# Autodesk Inventor assembly: Ensamblaje completo
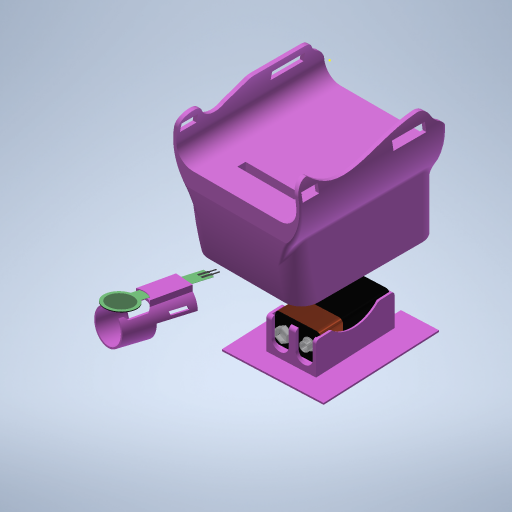
[picture p0: Inventor's stored thumbnail of the model, 512x512]
Saved by Autodesk Inventor 2024 (Build 280153000, 153)
## iProperties
Created: 2024-06-27
Part Number: Ensamblaje completo
Document SubType Name: Assembly
Designer: Valeria
Author: Valeria
## Documents named in this file (11)
- C:\Users\Valeria\Downloads\Ensamblaje completo.iam
- C:\Users\Valeria\Downloads\CASE batería.ipt
- C:\Users\Valeria\Downloads\9v-battery-11.snapshot.2\9v Duracell Battery Wyatt Sanders.ipt
- C:\Users\Valeria\Downloads\tapa ns (7).ipt
- C:\Users\Valeria\Downloads\coso tapa ns (3).ipt
- C:\Users\Valeria\Downloads\dedo ultimo xfa (1).ipt
- C:\Users\Valeria\Downloads\protoboard-400-pts-1.snapshot.5\proto_400\proto_400.ipt
- C:\Users\Valeria\Downloads\fsr402-1.snapshot.3\FSR 402\FSR 402.ipt
- C:\Users\Valeria\Downloads\arduino-nano-7.snapshot.2 (1)\arduino nano\arduino nano.ipt
- C:\Users\Valeria\Downloads\arduino-nano-7.snapshot.2 (1)\Green Detailed 5mm LED\Green Detailed 5mm LED.ipt
- C:\Users\Valeria\Downloads\arduino-nano-7.snapshot.2 (1)\Red Detailed 5mm LED\Red Detailed 5mm LED.ipt
## Components (10 placed, 10 different names)
1. CASE batería:1 — Coincidencia:1, Coincidencia:2, Coincidencia:3, Rígido:1
2. 9v Duracell Battery Wyatt Sanders:1 — Coincidencia:1, Coincidencia:2, Coincidencia:3
3. tapa ns (7):1 — Rígido:1
4. coso tapa ns (3):1 — Coincidencia:4, Coincidencia:7, Coincidencia:8, Coincidencia:9
5. dedo ultimo xfa (1):1 — Coincidencia:5
6. proto_400:1 — Coincidencia:4, Coincidencia:6
7. FSR 402:1 — Coincidencia:5
8. arduino nano:1 — Coincidencia:6
9. Green Detailed 5mm LED:1 — Coincidencia:7, Coincidencia:8
10. Red Detailed 5mm LED:1 — Coincidencia:9
## Relationships (10: Mate 9, WeldJoint 1)
- Coincidencia:1 [Mate]: CASE batería:1 ↔ 9v Duracell Battery Wyatt Sanders:1
- Coincidencia:2 [Mate]: CASE batería:1 ↔ 9v Duracell Battery Wyatt Sanders:1
- Coincidencia:3 [Mate]: CASE batería:1 ↔ 9v Duracell Battery Wyatt Sanders:1
- Rígido:1 [WeldJoint]: CASE batería:1 ↔ tapa ns (7):1
- Coincidencia:4 [Mate]: coso tapa ns (3):1 ↔ proto_400:1
- Coincidencia:5 [Mate]: dedo ultimo xfa (1):1 ↔ FSR 402:1
- Coincidencia:6 [Mate]: proto_400:1 ↔ arduino nano:1
- Coincidencia:7 [Mate]: coso tapa ns (3):1 ↔ Green Detailed 5mm LED:1
- Coincidencia:8 [Mate]: coso tapa ns (3):1 ↔ Green Detailed 5mm LED:1
- Coincidencia:9 [Mate]: coso tapa ns (3):1 ↔ Red Detailed 5mm LED:1
